# Autodesk Inventor assembly: PILLARSCELLCASE21700ASSEMBLY
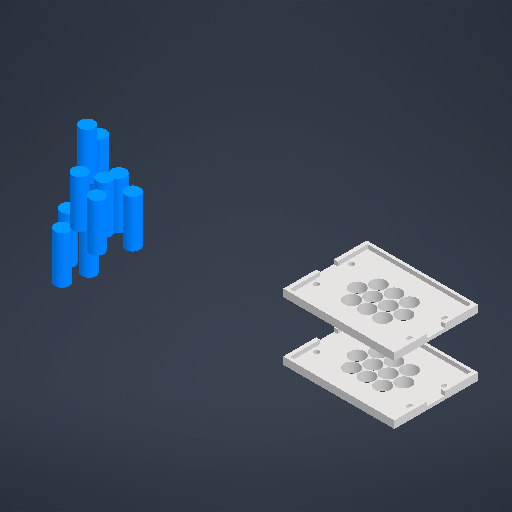
[picture p0: Inventor's stored thumbnail of the model, 512x512]
Saved by Autodesk Inventor 2025.2 (Build 292293000, 293)
## iProperties
Created: 2025-03-05
Part Number: PILLARSCELLCASE21700ASSEMBLY
Document SubType Name: Assembly
Designer: cbast
Author: cbast
## Documents named in this file (3)
- C:\Users\cbast\OneDrive\Documents\GitHub\Smart-Pack-for-Advanced-Research-and-Control\variations\Camden\V0.2\PILLARSCELLCASE21700ASSEMBLY.iam
- C:\Users\cbast\OneDrive\Documents\GitHub\Smart-Pack-for-Advanced-Research-and-Control\variations\Camden\V0.1\21700(Blue).ipt
- C:\Users\cbast\OneDrive\Documents\GitHub\Smart-Pack-for-Advanced-Research-and-Control\variations\Camden\V0.2\PILLARSCELLCASE21700.ipt
## Components (12 placed, 2 different names)
1. 21700(Blue):1
2. 21700(Blue):2
3. 21700(Blue):3
4. 21700(Blue):4
5. 21700(Blue):5
6. 21700(Blue):6
7. 21700(Blue):7
8. 21700(Blue):8
9. 21700(Blue):9
10. 21700(Blue):10
11. PILLARSCELLCASE21700:1 — Mate:1, Mate:2
12. PILLARSCELLCASE21700:2 — Mate:1, Mate:2
## Relationships (2: Mate 2)
- Mate:1: PILLARSCELLCASE21700:1 ↔ PILLARSCELLCASE21700:2
- Mate:2: PILLARSCELLCASE21700:1 ↔ PILLARSCELLCASE21700:2
